# Autodesk Inventor assembly: UPS_HAT_E
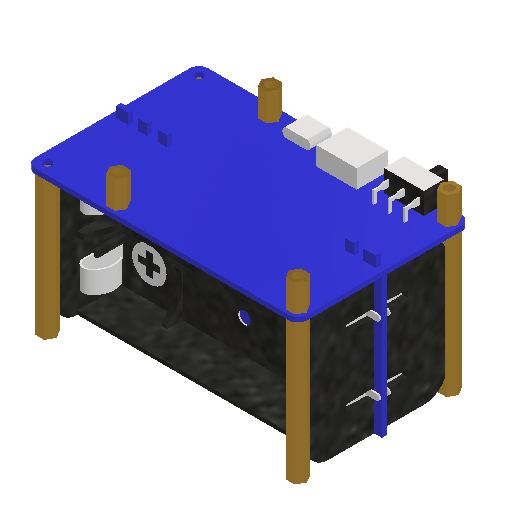
[picture p0: Inventor's stored thumbnail of the model, 512x512]
Saved by Autodesk Inventor 2025.2 (Build 292293000, 293)
## iProperties
Created: 2025-03-09
Part Number: UPS_HAT_E
Document SubType Name: Assembly
Designer: ahorat
Author: ahorat
## Documents named in this file (10)
- C:\Daten\Temp\R32EntrySystem\cad\UPS_HAT_E\UPS_HAT_E.iam
- C:\Daten\Temp\R32EntrySystem\cad\UPS_HAT_E\PCB_2.ipt
- C:\Daten\Temp\R32EntrySystem\cad\UPS_HAT_E\Holder_21700_Dual.iam
- C:\Daten\Temp\R32EntrySystem\cad\UPS_HAT_E\PCB_1.ipt
- C:\Daten\Temp\R32EntrySystem\cad\UPS_HAT_E\Switch.ipt
- C:\Daten\Temp\R32EntrySystem\cad\UPS_HAT_E\USB_A.ipt
- C:\Daten\Temp\R32EntrySystem\cad\UPS_HAT_E\USB_C.ipt
- C:\Daten\Temp\R32EntrySystem\cad\UPS_HAT_E\Spacer_9mm.ipt
- C:\Daten\Temp\R32EntrySystem\cad\UPS_HAT_E\Spacer_46mm.ipt
- C:\Daten\Temp\R32EntrySystem\cad\UPS_HAT_E\Spacer_9mm_screw.ipt
## Components (15 placed, 9 different names)
1. PCB_2:1 — Flush:2, Mate:2, Flush:3, Mate:3, Flush:4, Mate:4, Mate:5, Mate:6, Mate:7
2. Holder_21700_Dual:1 [sub-assembly] — Flush:2, Mate:2, Flush:3
3. Holder_21700_Dual:2 [sub-assembly] — Mate:3, Flush:4, Mate:4
4. PCB_1:1 — Mate:5, Mate:6, Mate:7, Mate:8, Mate:9, Mate:10, Mate:11, Flush:5, Flush:6, Mate:12, Flush:7, Flush:8, Insert:2, Insert:5, Insert:6, Insert:7, Insert:8, Insert:9, Insert:10, Insert:11
5. Switch:1 — Mate:8, Mate:9, Mate:10
6. USB_A:1 — Mate:11, Flush:5, Flush:6
7. USB_C:1 — Mate:12, Flush:7, Flush:8
8. Spacer_9mm_screw:1 — Insert:9
9. Spacer_46mm:1 — Insert:5
10. Spacer_9mm_screw:2 — Insert:2
11. Spacer_46mm:2 — Insert:6
12. Spacer_46mm:3 — Insert:7
13. Spacer_46mm:4 — Insert:8
14. Spacer_9mm:1 — Insert:10
15. Spacer_9mm:2 — Insert:11
## Relationships (26: Mate 11, Insert 8, Flush 7)
- Flush:2: PCB_2:1 ↔ Holder_21700_Dual:1
- Mate:2: PCB_2:1 ↔ Holder_21700_Dual:1
- Flush:3: PCB_2:1 ↔ Holder_21700_Dual:1
- Mate:3: PCB_2:1 ↔ Holder_21700_Dual:2
- Flush:4: PCB_2:1 ↔ Holder_21700_Dual:2
- Mate:4: PCB_2:1 ↔ Holder_21700_Dual:2
- Mate:5: PCB_2:1 ↔ PCB_1:1
- Mate:6: PCB_2:1 ↔ PCB_1:1
- Mate:7: PCB_2:1 ↔ PCB_1:1
- Mate:8: PCB_1:1 ↔ Switch:1
- Mate:9: PCB_1:1 ↔ Switch:1
- Mate:10: PCB_1:1 ↔ Switch:1
- Mate:11: PCB_1:1 ↔ USB_A:1
- Flush:5: PCB_1:1 ↔ USB_A:1
- Flush:6 (27 mm): PCB_1:1 ↔ USB_A:1
- Mate:12: PCB_1:1 ↔ USB_C:1
- Flush:7: PCB_1:1 ↔ USB_C:1
- Flush:8 (-45 mm): PCB_1:1 ↔ USB_C:1
- Insert:2: PCB_1:1 ↔ Spacer_9mm_screw:2
- Insert:5: PCB_1:1 ↔ Spacer_46mm:1
- Insert:6: PCB_1:1 ↔ Spacer_46mm:2
- Insert:7: PCB_1:1 ↔ Spacer_46mm:3
- Insert:8: PCB_1:1 ↔ Spacer_46mm:4
- Insert:9: PCB_1:1 ↔ Spacer_9mm_screw:1
- Insert:10: PCB_1:1 ↔ Spacer_9mm:1
- Insert:11: PCB_1:1 ↔ Spacer_9mm:2
